# Autodesk Inventor assembly: Roll_Fixation_Frame_8mm_Set_Backside
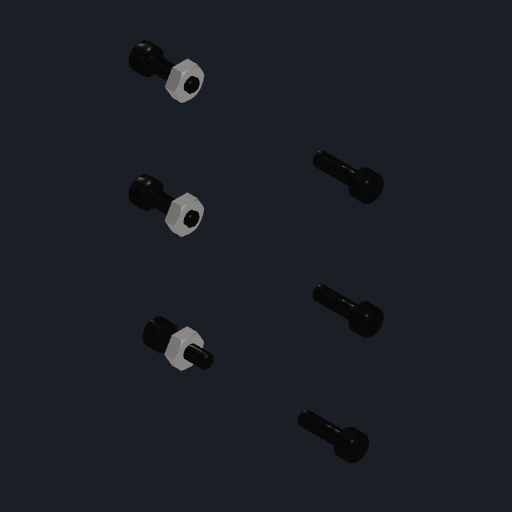
[picture p0: Inventor's stored thumbnail of the model, 512x512]
Saved by Autodesk Inventor 2024.3 (Build 283343000, 343)
## iProperties
Created: 2024-11-01
Part Number: Roll_Fixation_Frame_8mm_Set_Backside
Document SubType Name: Assembly
Designer: ASUS
Author: ASUS
## Documents named in this file (3)
- C:\Users\ASUS\Desktop\test\Screw_Set\Roll_Fixation_Frame_8mm_Set_Backside.iam
- C:\Users\ASUS\Desktop\test\v1_Frame\MISUMI\CSH-ST-M2_5-8.ipt
- C:\Users\ASUS\Desktop\test\v1_Frame\MISUMI\SLBNR2_5.ipt
## Components (9 placed, 2 different names)
1. CSH-ST-M2_5-8:1
2. SLBNR2_5:1
3. CSH-ST-M2_5-8:2
4. SLBNR2_5:2
5. CSH-ST-M2_5-8:3
6. CSH-ST-M2_5-8:4
7. SLBNR2_5:3
8. CSH-ST-M2_5-8:5
9. CSH-ST-M2_5-8:6
## Relationships (6: Mate 3, Insert 3)
- [Mate]: SLBNR2_5:2 ↔ CSH-ST-M2_5-8:3
- [Mate]: SLBNR2_5:1 ↔ CSH-ST-M2_5-8:2
- [Insert] (2.5 mm): SLBNR2_5:2 ↔ CSH-ST-M2_5-8:3
- [Insert] (5.25 mm): SLBNR2_5:1 ↔ CSH-ST-M2_5-8:2
- [Mate]: SLBNR2_5:3 ↔ CSH-ST-M2_5-8:5
- [Insert] (5.25 mm): SLBNR2_5:3 ↔ CSH-ST-M2_5-8:5
## Named parameters: d37_d804 = 0 mm, d38_d32 = 5.25 mm
